# Autodesk Inventor assembly: BallBearing
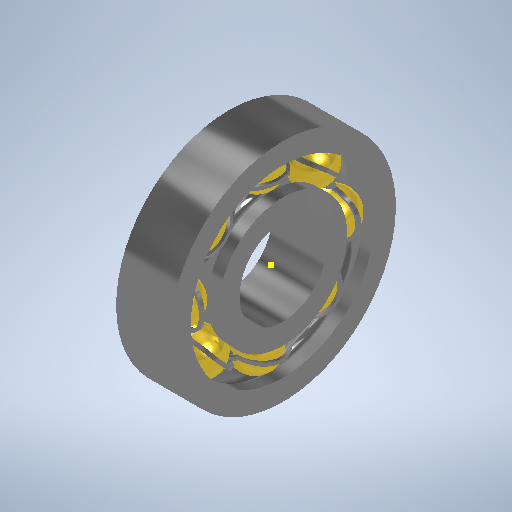
[picture p0: Inventor's stored thumbnail of the model, 512x512]
Saved by Autodesk Inventor 2025.1 (Build 291241000, 241)
## iProperties
Created: 2024-08-09
Part Number: BallBearing
Document SubType Name: Assembly
Designer: vedan
Author: vedan
## Documents named in this file (6)
- C:\Users\vedan\OneDrive\Desktop\CAD\BallBearing.iam
- C:\Users\vedan\OneDrive\Desktop\CAD\Ball.ipt
- C:\Users\vedan\OneDrive\Desktop\CAD\Inner ring.ipt
- C:\Users\vedan\OneDrive\Desktop\CAD\Outer ring.ipt
- C:\Users\vedan\OneDrive\Desktop\CAD\Crown.ipt
- C:\Users\vedan\OneDrive\Desktop\CAD\Crown_MIR2.ipt
## Components (12 placed, 5 different names)
1. Crown:1 — Mate:3, Mate:4, Mate:5
2. Inner ring:1 — Mate:1, Mate:2, Tangent:2, Mate:4
3. Outer ring:1 — Mate:1, Mate:2, Tangent:1, Mate:3, Mate:6
4. Crown_MIR2:1 — Mate:6, Tangent:3
5. Ball:1 — Tangent:1, Tangent:2, Mate:5, Tangent:3
6. Ball:2
7. Ball:3
8. Ball:4
9. Ball:5
10. Ball:6
11. Ball:7
12. Ball:8
## Component patterns: (8 elements, first: Ball:1)
## Relationships (9: Mate 6, Tangent 3)
- Mate:1: Inner ring:1 ↔ Outer ring:1
- Mate:2: Inner ring:1 ↔ Outer ring:1
- Tangent:1: Outer ring:1 ↔ Ball:1
- Tangent:2: Inner ring:1 ↔ Ball:1
- Mate:3: Crown:1 ↔ Outer ring:1
- Mate:4: Crown:1 ↔ Inner ring:1
- Mate:5: Crown:1 ↔ Ball:1
- Mate:6: Outer ring:1 ↔ Crown_MIR2:1
- Tangent:3: Crown_MIR2:1 ↔ Ball:1
